# Autodesk Inventor assembly: board_user.1
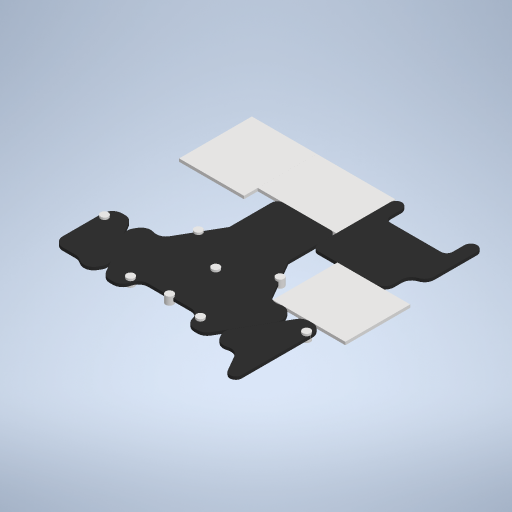
[picture p0: Inventor's stored thumbnail of the model, 512x512]
Saved by Autodesk Inventor 2024.1 (Build 281209000, 209)
## iProperties
Created: 2025-04-13
Part Number: board_user.1
Document SubType Name: Assembly
Designer: hibik
Author: hibik
## Documents named in this file (3)
- C:\Users\hibik\Documents\Robomech\RESCUE\ORCA\hard\board\CORE\board_user.1.iam
- C:\Users\hibik\Documents\Robomech\RESCUE\ORCA\hard\board\CORE\board_outline.iam
- C:\Users\hibik\Documents\Robomech\RESCUE\ORCA\hard\board\CORE\CORE_set_user.1_.ipt
## Components (2 placed, 2 different names)
1. board_outline:1 [sub-assembly]
2. CORE_set_user.1_:1 — フラッシュ:1, フラッシュ:2, フラッシュ:3
## Relationships (3: Flush 3)
- フラッシュ:1 [Flush]: CORE_set_user.1_:1
- フラッシュ:2 [Flush]: CORE_set_user.1_:1
- フラッシュ:3 [Flush]: CORE_set_user.1_:1
